# Autodesk Inventor assembly: platform
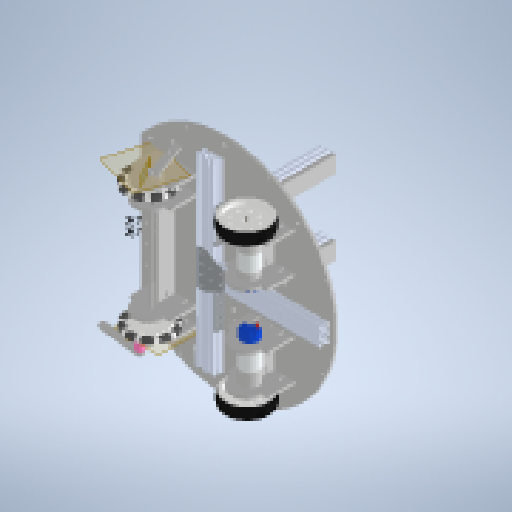
[picture p0: Inventor's stored thumbnail of the model, 512x512]
Saved by Autodesk Inventor 2023 (Build 270158000, 158)
## iProperties
Created: 2023-03-13
Part Number: platform
Document SubType Name: Assembly
Designer: User
Author: User
## Documents named in this file (35)
- \\sch239.net\UserHomes\Students\other\baranovaem\cheburashka\Cheburashka-main\Cheburashka_construction\platform\platform.iam
- \\sch239.net\UserHomes\Students\other\baranovaem\cheburashka\Cheburashka-main\Cheburashka_construction\platform\Osn. platform.ipt
- \\sch239.net\UserHomes\Students\other\baranovaem\cheburashka\Cheburashka-main\Cheburashka_construction\platform\motor1.ipt
- \\sch239.net\UserHomes\Students\other\baranovaem\cheburashka\Cheburashka-main\Cheburashka_construction\platform\motor2.ipt
- \\sch239.net\UserHomes\Students\other\baranovaem\cheburashka\Cheburashka-main\Cheburashka_construction\platform\motor3.ipt
- \\sch239.net\UserHomes\Students\other\baranovaem\cheburashka\Cheburashka-main\Cheburashka_construction\platform\wheel1.ipt
- \\sch239.net\UserHomes\Students\other\baranovaem\cheburashka\Cheburashka-main\Cheburashka_construction\platform\44260_txm torquenado dc motor_MIR2.ipt
- \\sch239.net\UserHomes\Students\other\baranovaem\cheburashka\Cheburashka-main\Cheburashka_construction\platform\36466_txm-4 inch omni wheel.ipt
- \\sch239.net\UserHomes\Students\other\baranovaem\cheburashka\Cheburashka-main\Cheburashka_construction\platform\39055_txm-4 inch wheel_MIR1.ipt
- \\sch239.net\UserHomes\Students\other\baranovaem\cheburashka\Cheburashka-main\Cheburashka_construction\platform\motor1_MIR3.ipt
- \\sch239.net\UserHomes\Students\other\baranovaem\cheburashka\Cheburashka-main\Cheburashka_construction\platform\motor2_MIR3.ipt
- \\sch239.net\UserHomes\Students\other\baranovaem\cheburashka\Cheburashka-main\Cheburashka_construction\platform\motor3_MIR3.ipt
- \\sch239.net\UserHomes\Students\other\baranovaem\cheburashka\Cheburashka-main\Cheburashka_construction\platform\44260_txm torquenado dc motor_MIR2_MIR.ipt
- \\sch239.net\UserHomes\Students\other\baranovaem\cheburashka\Cheburashka-main\Cheburashka_construction\platform\wheel1_MIR.ipt
- \\sch239.net\UserHomes\Students\other\baranovaem\cheburashka\Cheburashka-main\Cheburashka_construction\platform\36466_txm-4 inch omni wheel_MIR2.ipt
- \\sch239.net\UserHomes\Students\other\baranovaem\cheburashka\Cheburashka-main\Cheburashka_construction\platform\39055_txm-4 inch wheel_MIR1_MIR.ipt
- \\sch239.net\UserHomes\Students\other\baranovaem\cheburashka\Cheburashka-main\Cheburashka_construction\platform\кривошип.ipt
- \\sch239.net\UserHomes\Students\other\baranovaem\cheburashka\Cheburashka-main\Cheburashka_construction\platform\ось колес2.ipt
- \\sch239.net\UserHomes\Students\other\baranovaem\cheburashka\Cheburashka-main\Cheburashka_construction\platform\akfytw2.ipt
- \\sch239.net\UserHomes\Students\other\baranovaem\cheburashka\Cheburashka-main\Cheburashka_construction\platform\подшипник2.ipt
- \\sch239.net\UserHomes\Students\other\baranovaem\cheburashka\Cheburashka-main\Cheburashka_construction\platform\шатун22.ipt
- \\sch239.net\UserHomes\Students\other\baranovaem\cheburashka\Cheburashka-main\Cheburashka_construction\platform\канал_проводов.ipt
- \\sch239.net\UserHomes\Students\other\baranovaem\cheburashka\Cheburashka-main\Cheburashka_construction\platform\обр_профиль.ipt
- \\sch239.net\UserHomes\Students\other\baranovaem\cheburashka\Cheburashka-main\Cheburashka_construction\platform\обр_профиль2.ipt
- \\sch239.net\UserHomes\Students\other\baranovaem\cheburashka\Cheburashka-main\Cheburashka_construction\platform\8bc17c1464c21f56fb2a3979b7c6b729.ipt
- \\sch239.net\UserHomes\Students\other\baranovaem\cheburashka\Cheburashka-main\Cheburashka_construction\platform\L72-T_soedinitel-60kh80.ipt
- \\sch239.net\UserHomes\Students\other\baranovaem\cheburashka\Cheburashka-main\Cheburashka_construction\platform\ребро.ipt
- \\sch239.net\UserHomes\Students\other\baranovaem\cheburashka\Cheburashka-main\Cheburashka_construction\platform\стенд.ipt
- \\sch239.net\UserHomes\Students\other\baranovaem\cheburashka\Cheburashka-main\Cheburashka_construction\platform\Raspberry Pi Camera Stand - 274111\files\camera_back_cover_v002.ipt
- \\sch239.net\UserHomes\Students\other\baranovaem\cheburashka\Cheburashka-main\Cheburashka_construction\platform\Raspberry Pi Camera Stand - 274111\files\camera_front_box_v003.ipt
- \\sch239.net\UserHomes\Students\other\baranovaem\cheburashka\Cheburashka-main\Cheburashka_construction\platform\кривошип_MIR.ipt
- \\sch239.net\UserHomes\Students\other\baranovaem\cheburashka\Cheburashka-main\Cheburashka_construction\platform\akfytw2_MIR.ipt
- \\sch239.net\UserHomes\Students\other\baranovaem\cheburashka\Cheburashka-main\Cheburashka_construction\platform\шатун22_MIR.ipt
- \\sch239.net\UserHomes\Students\other\baranovaem\cheburashka\Cheburashka-main\Cheburashka_construction\platform\4ad8d019baf454c6bbd45c2c6ffb6783.ipt
- \\sch239.net\UserHomes\Students\other\baranovaem\cheburashka\Cheburashka-main\Cheburashka_construction\platform\гриб.ipt
## Components (43 placed, 34 different names)
1. Osn. platform:1 — Совмещение:129, Совмещение:130, Совмещение:131, Совмещение:132, Совмещение:133, Совмещение:137, Совмещение:138, Совмещение:155, Совмещение:158, Совмещение:178, Совмещение:181, Совмещение:182, Совмещение:183, Совмещение:184, Совмещение:185, Совмещение:186, Совмещение:192, Совмещение:193, Совмещение:194, Совмещение:195, Совмещение:196, Совмещение:197, Совмещение:198, Совмещение:213, Совмещение:214, Совмещение:215, Совмещение:216, Совмещение:217, Совмещение:218, Совмещение:219, Совмещение:230, Совмещение:231, Совмещение:232, Совмещение:233
2. motor1:1 — Совмещение:181, Совмещение:182
3. motor2:1 — Совмещение:232, Совмещение:233
4. motor3:1 — Совмещение:230, Совмещение:231
5. 44260_txm torquenado dc motor_MIR2:1 — Совмещение:21
6. wheel1:1 — Совмещение:101, Совмещение:185, Совмещение:186
7. 36466_txm-4 inch omni wheel:1
8. 39055_txm-4 inch wheel_MIR1:1 — Совмещение:21
9. motor1_MIR3:1 — Совмещение:183, Совмещение:184
10. motor2_MIR3:1 — Совмещение:148
11. motor3_MIR3:1 — Совмещение:109, Совмещение:110, Совмещение:111
12. 44260_txm torquenado dc motor_MIR2_MIR:1 — Совмещение:28, Совмещение:109, Совмещение:110, Совмещение:148
13. wheel1_MIR:1 — Совмещение:189, Совмещение:192, Совмещение:197, Совмещение:198, Совмещение:228
14. wheel1_MIR:2 — Совмещение:195, Совмещение:196
15. 36466_txm-4 inch omni wheel_MIR2:1 — Совмещение:229
16. 39055_txm-4 inch wheel_MIR1_MIR:1 — Совмещение:28, Совмещение:111
17. кривошип:1 — Совмещение:90, Совмещение:91, Совмещение:92, Совмещение:93, Совмещение:96
18. ось колес2:1 — Совмещение:228, Совмещение:229
19. akfytw2:1 — Совмещение:90, Совмещение:91, Совмещение:101
20. подшипник2:1 — Совмещение:92, Совмещение:93, Совмещение:94
21. подшипник2:2 — Совмещение:94, Совмещение:95
22. шатун22:1 — Совмещение:95, Совмещение:96, Совмещение:225, Совмещение:226, Совмещение:227
23. канал_проводов:1 — Совмещение:213, Совмещение:214
24. канал_проводов:2 — Совмещение:215, Совмещение:216
25. обр_профиль:1 — Совмещение:129, Совмещение:130, Совмещение:131, Совмещение:179, Совмещение:206, Совмещение:207, Совмещение:208, Совмещение:210
26. обр_профиль:2 — Совмещение:132, Совмещение:133, Совмещение:135, Совмещение:136, Совмещение:157, Совмещение:212
27. обр_профиль2:1 — Совмещение:135, Совмещение:136, Совмещение:139, Совмещение:204, Совмещение:205, Совмещение:209, Совмещение:211
28. обр_профиль:3 — Совмещение:137, Совмещение:138, Совмещение:139
29. 8bc17c1464c21f56fb2a3979b7c6b729:1 — Совмещение:155, Совмещение:206, Совмещение:207
30. 8bc17c1464c21f56fb2a3979b7c6b729:2 — Совмещение:157, Совмещение:158
31. L72-T_soedinitel-60kh80:1 — Совмещение:209, Совмещение:210
32. L72-T_soedinitel-60kh80:2 — Совмещение:211, Совмещение:212
33. L72-T_soedinitel-60kh80:3 — Совмещение:204, Совмещение:205
34. ребро:1 — Совмещение:201, Совмещение:202, Совмещение:203
35. camera_back_cover_v002:1 — Совмещение:222, Совмещение:223, Совмещение:224
36. camera_front_box_v003:1 — Совмещение:220, Совмещение:221, Совмещение:222, Совмещение:223, Совмещение:224
37. кривошип_MIR:1 — Совмещение:190, Совмещение:191, Совмещение:199, Совмещение:200
38. akfytw2_MIR:1 — Совмещение:189, Совмещение:190, Совмещение:191
39. шатун22_MIR:1 — Совмещение:199, Совмещение:200
40. 4ad8d019baf454c6bbd45c2c6ffb6783:1 — Совмещение:178, Совмещение:179, Совмещение:208
41. wheel1:2 — Совмещение:193, Совмещение:194, Совмещение:201, Совмещение:202, Совмещение:203
42. стенд:1 — Совмещение:217, Совмещение:218, Совмещение:219, Совмещение:220, Совмещение:221
43. гриб:1 — Совмещение:225, Совмещение:226, Совмещение:227
## Relationships (80: Mate 80)
- Совмещение:21 [Mate]: 44260_txm torquenado dc motor_MIR2:1 ↔ 39055_txm-4 inch wheel_MIR1:1
- Совмещение:28 [Mate]: 44260_txm torquenado dc motor_MIR2_MIR:1 ↔ 39055_txm-4 inch wheel_MIR1_MIR:1
- Совмещение:90 [Mate]: кривошип:1 ↔ akfytw2:1
- Совмещение:91 [Mate]: кривошип:1 ↔ akfytw2:1
- Совмещение:92 [Mate]: кривошип:1 ↔ подшипник2:1
- Совмещение:93 [Mate]: кривошип:1 ↔ подшипник2:1
- Совмещение:94 [Mate]: подшипник2:1 ↔ подшипник2:2
- Совмещение:95 [Mate]: подшипник2:2 ↔ шатун22:1
- Совмещение:96 [Mate] (2 mm): кривошип:1 ↔ шатун22:1
- Совмещение:101 [Mate]: wheel1:1 ↔ akfytw2:1
- Совмещение:109 [Mate]: motor3_MIR3:1 ↔ 44260_txm torquenado dc motor_MIR2_MIR:1
- Совмещение:110 [Mate]: motor3_MIR3:1 ↔ 44260_txm torquenado dc motor_MIR2_MIR:1
- Совмещение:111 [Mate] (5 mm): motor3_MIR3:1 ↔ 39055_txm-4 inch wheel_MIR1_MIR:1
- Совмещение:129 [Mate]: Osn. platform:1 ↔ обр_профиль:1
- Совмещение:130 [Mate]: Osn. platform:1 ↔ обр_профиль:1
- Совмещение:131 [Mate]: Osn. platform:1 ↔ обр_профиль:1
- Совмещение:132 [Mate]: Osn. platform:1 ↔ обр_профиль:2
- Совмещение:133 [Mate]: Osn. platform:1 ↔ обр_профиль:2
- Совмещение:135 [Mate] (99.253 mm): обр_профиль:2 ↔ обр_профиль2:1
- Совмещение:136 [Mate]: обр_профиль:2 ↔ обр_профиль2:1
- Совмещение:137 [Mate]: Osn. platform:1 ↔ обр_профиль:3
- Совмещение:138 [Mate] (4.43 mm): Osn. platform:1 ↔ обр_профиль:3
- Совмещение:139 [Mate]: обр_профиль2:1 ↔ обр_профиль:3
- Совмещение:148 [Mate]: motor2_MIR3:1 ↔ 44260_txm torquenado dc motor_MIR2_MIR:1
- Совмещение:155 [Mate]: Osn. platform:1 ↔ 8bc17c1464c21f56fb2a3979b7c6b729:1
- Совмещение:157 [Mate]: обр_профиль:2 ↔ 8bc17c1464c21f56fb2a3979b7c6b729:2
- Совмещение:158 [Mate]: Osn. platform:1 ↔ 8bc17c1464c21f56fb2a3979b7c6b729:2
- Совмещение:178 [Mate]: Osn. platform:1 ↔ 4ad8d019baf454c6bbd45c2c6ffb6783:1
- Совмещение:179 [Mate]: обр_профиль:1 ↔ 4ad8d019baf454c6bbd45c2c6ffb6783:1
- Совмещение:181 [Mate]: Osn. platform:1 ↔ motor1:1
- Совмещение:182 [Mate]: Osn. platform:1 ↔ motor1:1
- Совмещение:183 [Mate]: Osn. platform:1 ↔ motor1_MIR3:1
- Совмещение:184 [Mate]: Osn. platform:1 ↔ motor1_MIR3:1
- Совмещение:185 [Mate]: Osn. platform:1 ↔ wheel1:1
- Совмещение:186 [Mate]: Osn. platform:1 ↔ wheel1:1
- Совмещение:189 [Mate]: wheel1_MIR:1 ↔ akfytw2_MIR:1
- Совмещение:190 [Mate]: кривошип_MIR:1 ↔ akfytw2_MIR:1
- Совмещение:191 [Mate]: кривошип_MIR:1 ↔ akfytw2_MIR:1
- Совмещение:192 [Mate]: Osn. platform:1 ↔ wheel1_MIR:1
- Совмещение:193 [Mate]: Osn. platform:1 ↔ wheel1:2
- Совмещение:194 [Mate]: Osn. platform:1 ↔ wheel1:2
- Совмещение:195 [Mate]: Osn. platform:1 ↔ wheel1_MIR:2
- Совмещение:196 [Mate]: Osn. platform:1 ↔ wheel1_MIR:2
- Совмещение:197 [Mate]: Osn. platform:1 ↔ wheel1_MIR:1
- Совмещение:198 [Mate]: Osn. platform:1 ↔ wheel1_MIR:1
- Совмещение:199 [Mate] (4 mm): кривошип_MIR:1 ↔ шатун22_MIR:1
- Совмещение:200 [Mate]: кривошип_MIR:1 ↔ шатун22_MIR:1
- Совмещение:201 [Mate]: ребро:1 ↔ wheel1:2
- Совмещение:202 [Mate]: ребро:1 ↔ wheel1:2
- Совмещение:203 [Mate]: ребро:1 ↔ wheel1:2
- Совмещение:204 [Mate]: обр_профиль2:1 ↔ L72-T_soedinitel-60kh80:3
- Совмещение:205 [Mate]: обр_профиль2:1 ↔ L72-T_soedinitel-60kh80:3
- Совмещение:206 [Mate]: обр_профиль:1 ↔ 8bc17c1464c21f56fb2a3979b7c6b729:1
- Совмещение:207 [Mate]: обр_профиль:1 ↔ 8bc17c1464c21f56fb2a3979b7c6b729:1
- Совмещение:208 [Mate]: обр_профиль:1 ↔ 4ad8d019baf454c6bbd45c2c6ffb6783:1
- Совмещение:209 [Mate]: обр_профиль2:1 ↔ L72-T_soedinitel-60kh80:1
- Совмещение:210 [Mate]: обр_профиль:1 ↔ L72-T_soedinitel-60kh80:1
- Совмещение:211 [Mate]: обр_профиль2:1 ↔ L72-T_soedinitel-60kh80:2
- Совмещение:212 [Mate]: обр_профиль:2 ↔ L72-T_soedinitel-60kh80:2
- Совмещение:213 [Mate]: Osn. platform:1 ↔ канал_проводов:1
- Совмещение:214 [Mate]: Osn. platform:1 ↔ канал_проводов:1
- Совмещение:215 [Mate]: Osn. platform:1 ↔ канал_проводов:2
- Совмещение:216 [Mate]: Osn. platform:1 ↔ канал_проводов:2
- Совмещение:217 [Mate]: Osn. platform:1 ↔ стенд:1
- Совмещение:218 [Mate]: Osn. platform:1 ↔ стенд:1
- Совмещение:219 [Mate]: Osn. platform:1 ↔ стенд:1
- Совмещение:220 [Mate]: camera_front_box_v003:1 ↔ стенд:1
- Совмещение:221 [Mate]: camera_front_box_v003:1 ↔ стенд:1
- Совмещение:222 [Mate]: camera_back_cover_v002:1 ↔ camera_front_box_v003:1
- Совмещение:223 [Mate]: camera_back_cover_v002:1 ↔ camera_front_box_v003:1
- Совмещение:224 [Mate]: camera_back_cover_v002:1 ↔ camera_front_box_v003:1
- Совмещение:225 [Mate]: шатун22:1 ↔ гриб:1
- Совмещение:226 [Mate]: шатун22:1 ↔ гриб:1
- Совмещение:227 [Mate] (-1.6 mm): шатун22:1 ↔ гриб:1
- Совмещение:228 [Mate]: wheel1_MIR:1 ↔ ось колес2:1
- Совмещение:229 [Mate]: 36466_txm-4 inch omni wheel_MIR2:1 ↔ ось колес2:1
- Совмещение:230 [Mate]: Osn. platform:1 ↔ motor3:1
- Совмещение:231 [Mate]: Osn. platform:1 ↔ motor3:1
- Совмещение:232 [Mate]: Osn. platform:1 ↔ motor2:1
- Совмещение:233 [Mate]: Osn. platform:1 ↔ motor2:1
